# Autodesk Inventor assembly: project slot
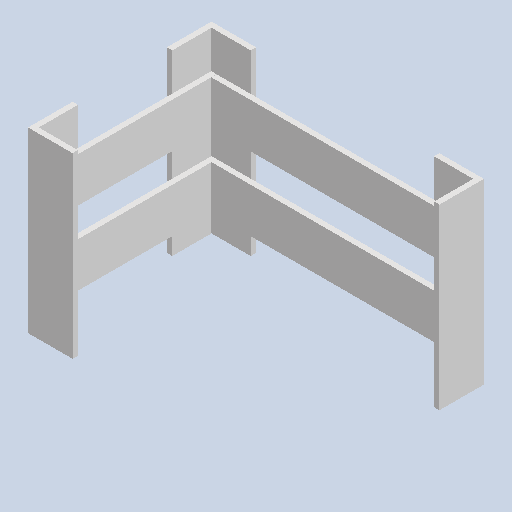
[picture p0: Inventor's stored thumbnail of the model, 512x512]
Saved by Autodesk Inventor 2025.2 (Build 292293000, 293)
## iProperties
Created: 2025-02-04
Part Number: project slot
Document SubType Name: Assembly
Designer: nandu
Author: nandu
## Documents named in this file (4)
- C:\Users\Khushal\Documents\College\Sem 4\TA212\Project_Latest\project slot.iam
- C:\Users\Khushal\Documents\College\Sem 4\TA212\Project_Latest\slot pillars.ipt
- C:\Users\Khushal\Documents\College\Sem 4\TA212\Project_Latest\slot small.ipt
- C:\Users\Khushal\Documents\College\Sem 4\TA212\Project_Latest\slot big.ipt
## Components (5 placed, 3 different names)
1. slot pillars:1 — Mate:1, Mate:2, Mate:3, Mate:4
2. slot small:1 — Mate:2
3. slot small:2 — Mate:1
4. slot big:1 — Mate:3
5. slot big:2 — Mate:4
## Relationships (4: Mate 4)
- Mate:1: slot pillars:1 ↔ slot small:2
- Mate:2: slot pillars:1 ↔ slot small:1
- Mate:3: slot pillars:1 ↔ slot big:1
- Mate:4: slot pillars:1 ↔ slot big:2
